# Autodesk Inventor assembly: Hopper Idler assy (mirrored)
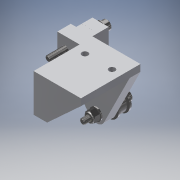
[picture p0: Inventor's stored thumbnail of the model, 180x180]
Saved by Autodesk Inventor 2018 (Build 220112000, 112)
## iProperties
Created: 2017-09-20
Part Number: Hopper Idler assy (mirrored)
Document SubType Name: Assembly
Designer: Gabriel Smolnycki
Author: Gabriel Smolnycki
## Documents named in this file (9)
- E:\planb\mechanics\V1INV\Subassemblies\Hopper Idler assy (mirrored).iam
- E:\planb\mechanics\V1INV\Hopper\Hopper Idler (mirrored).ipt
- E:\planb\mechanics\V1INV\Hopper\Hopper Smooth Rod Clamp.ipt
- E:\planb\mechanics\V1INV\Hardware\M4 SS Washer.ipt
- E:\planb\mechanics\V1INV\Hardware\M4x40 SS SHCS.ipt
- E:\planb\mechanics\V1INV\Hardware\M4 SS Locknut.ipt
- E:\planb\mechanics\V1INV\Hardware\M4x30 SS SHCS.ipt
- E:\planb\mechanics\V1INV\Hardware\M5 SS Fender Washer.ipt
- E:\planb\mechanics\V1INV\Hardware\4x13 SS Ball Bearing (7804K103).ipt
## Components (17 placed, 8 different names)
1. Hopper Idler (mirrored):1 — Insert:1, Insert:2, Insert:19, Insert:20
2. Hopper Smooth Rod Clamp:1 — Insert:3, Insert:4, Insert:5, Insert:6
3. Hopper Smooth Rod Clamp:2 — Insert:1, Insert:2, Insert:3, Insert:4
4. M4 SS Washer:1 — Insert:5, Insert:7
5. M4 SS Washer:2 — Insert:6, Insert:8
6. M4x40 SS SHCS:1 — Insert:8
7. M4x40 SS SHCS:2 — Insert:7
8. M4x30 SS SHCS:1 — Insert:12
9. M4 SS Washer:3 — Insert:12, Insert:13
10. M4 SS Washer:4 — Insert:14, Insert:15
11. M4 SS Washer:5 — Insert:16, Insert:17
12. M4 SS Washer:6 — Insert:18, Insert:19
13. M5 SS Fender Washer:1 — Insert:13, Insert:14
14. M5 SS Fender Washer:2 — Insert:17, Insert:18
15. M4 SS Washer:7 — Insert:20, Insert:21
16. M4 SS Locknut:3 — Insert:21
17. 4x13 SS Ball Bearing (7804K103):1 — Insert:15, Insert:16
## Relationships (18: Insert 18)
- Insert:1: Hopper Idler (mirrored):1 ↔ Hopper Smooth Rod Clamp:2
- Insert:2: Hopper Idler (mirrored):1 ↔ Hopper Smooth Rod Clamp:2
- Insert:3: Hopper Smooth Rod Clamp:1 ↔ Hopper Smooth Rod Clamp:2
- Insert:4: Hopper Smooth Rod Clamp:1 ↔ Hopper Smooth Rod Clamp:2
- Insert:5: Hopper Smooth Rod Clamp:1 ↔ M4 SS Washer:1
- Insert:6: Hopper Smooth Rod Clamp:1 ↔ M4 SS Washer:2
- Insert:7: M4 SS Washer:1 ↔ M4x40 SS SHCS:2
- Insert:8: M4 SS Washer:2 ↔ M4x40 SS SHCS:1
- Insert:12: M4x30 SS SHCS:1 ↔ M4 SS Washer:3
- Insert:13: M4 SS Washer:3 ↔ M5 SS Fender Washer:1
- Insert:14: M4 SS Washer:4 ↔ M5 SS Fender Washer:1
- Insert:15: M4 SS Washer:4 ↔ 4x13 SS Ball Bearing (7804K103):1
- Insert:16: M4 SS Washer:5 ↔ 4x13 SS Ball Bearing (7804K103):1
- Insert:17: M4 SS Washer:5 ↔ M5 SS Fender Washer:2
- Insert:18: M4 SS Washer:6 ↔ M5 SS Fender Washer:2
- Insert:19: Hopper Idler (mirrored):1 ↔ M4 SS Washer:6
- Insert:20: Hopper Idler (mirrored):1 ↔ M4 SS Washer:7
- Insert:21: M4 SS Washer:7 ↔ M4 SS Locknut:3
